# Autodesk Inventor assembly: Turret_Assem
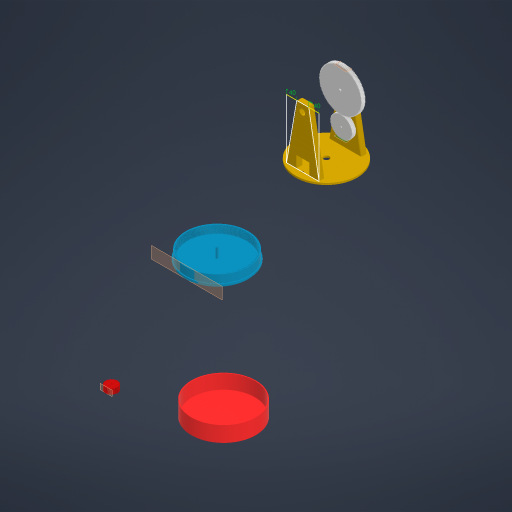
[picture p0: Inventor's stored thumbnail of the model, 512x512]
Saved by Autodesk Inventor 2023 (Build 270158030, 158C)
## iProperties
Created: 2022-05-13
Part Number: Turret_Assem
Document SubType Name: Assembly
Designer: jayso
Author: jayso
## Documents named in this file (8)
- C:\Users\jayso\Desktop\Nerf-Turret\CAD\Turret_Assem.iam
- C:\Users\jayso\Desktop\Nerf-Turret\CAD\electronics-base.ipt
- C:\Users\jayso\Desktop\Nerf-Turret\CAD\electronics-cover.ipt
- C:\Users\jayso\Desktop\Nerf-Turret\CAD\y-axis-gear.ipt
- C:\Users\jayso\Desktop\Nerf-Turret\CAD\x-axis-gear.ipt
- C:\Users\jayso\Desktop\Nerf-Turret\CAD\turret-base.ipt
- C:\Users\jayso\Desktop\Nerf-Turret\CAD\shooter-right-shaft-attach.ipt
- C:\Users\jayso\Desktop\Nerf-Turret\CAD\Turret_Assem\Design Accelerator\Bearing1.iam
## Components (7 placed, 7 different names)
1. electronics-base:1
2. electronics-cover:1
3. y-axis-gear:1
4. x-axis-gear:1
5. turret-base:1 — Mate:1, Rigid:1
6. Bearing:1 [sub-assembly] — Mate:1
7. shooter-right-shaft-attach:1 — Rigid:1
## Relationships (2: Mate 1, WeldJoint 1)
- Mate:1: turret-base:1 ↔ Bearing:1
- Rigid:1 [WeldJoint] (20.6375 mm): turret-base:1 ↔ shooter-right-shaft-attach:1
